# Autodesk Inventor assembly: Ribbon_Twitter
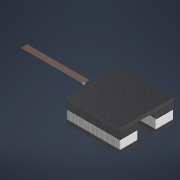
[picture p0: Inventor's stored thumbnail of the model, 180x180]
Saved by Autodesk Inventor 2022 (Build 260153070, 153G)
## iProperties
Created: 2022-02-01
Part Number: Ribbon_Twitter
Document SubType Name: Assembly
Designer: kalugin_a
Author: kalugin_a
## Documents named in this file (7)
- C:\Users\kalugin_a\Documents\Inventor\TUTO\MELAS\Workspace\Ribbon_Twitter.iam
- C:\Users\kalugin_a\Documents\Inventor\TUTO\MELAS\Workspace\NS.ipt
- C:\Users\kalugin_a\Documents\Inventor\TUTO\MELAS\Workspace\plate.ipt
- C:\Users\kalugin_a\Documents\Inventor\TUTO\MELAS\Workspace\Plate1.ipt
- C:\Users\kalugin_a\Documents\Inventor\TUTO\MELAS\Workspace\flange.ipt
- C:\Users\kalugin_a\Documents\Inventor\TUTO\MELAS\Workspace\Mwire.ipt
- C:\Users\kalugin_a\Documents\Inventor\TUTO\MELAS\Workspace\ribbon.ipt
## Components (11 placed, 6 different names)
1. NS:1 — Заподлицо:9, Заподлицо:10, Совмещение:5, Совмещение:7, Совмещение:8, Заподлицо:13, Заподлицо:14
2. NS:2 — Совмещение:6, Заподлицо:11, Заподлицо:12, Совмещение:9, Заподлицо:15, Заподлицо:16
3. plate:1 — Заподлицо:1, Заподлицо:2, Совмещение:1, Заподлицо:5, Заподлицо:6, Совмещение:3
4. Plate1:1 — Заподлицо:5, Заподлицо:6, Совмещение:3, Заподлицо:7, Совмещение:4, Заподлицо:8, Заподлицо:10
5. Plate1:2 — Заподлицо:1, Заподлицо:2, Совмещение:1, Заподлицо:3, Заподлицо:4, Совмещение:2, Заподлицо:12
6. Plate1:3 — Заподлицо:7, Совмещение:4, Заподлицо:8, Заподлицо:9, Совмещение:5
7. Plate1:4 — Заподлицо:3, Заподлицо:4, Совмещение:2, Совмещение:6, Заподлицо:11
8. flange:1 — Совмещение:7
9. Mwire:1 — Совмещение:8, Заподлицо:13, Заподлицо:14
10. Mwire:2 — Совмещение:9, Заподлицо:15, Заподлицо:16
11. ribbon:1
## Relationships (25: Flush 16, Mate 9)
- Заподлицо:1 [Flush]: plate:1 ↔ Plate1:2
- Заподлицо:2 [Flush]: plate:1 ↔ Plate1:2
- Совмещение:1 [Mate]: plate:1 ↔ Plate1:2
- Заподлицо:3 [Flush]: Plate1:2 ↔ Plate1:4
- Заподлицо:4 [Flush]: Plate1:2 ↔ Plate1:4
- Совмещение:2 [Mate]: Plate1:2 ↔ Plate1:4
- Заподлицо:5 [Flush]: plate:1 ↔ Plate1:1
- Заподлицо:6 [Flush]: plate:1 ↔ Plate1:1
- Совмещение:3 [Mate]: plate:1 ↔ Plate1:1
- Заподлицо:7 [Flush]: Plate1:1 ↔ Plate1:3
- Совмещение:4 [Mate]: Plate1:1 ↔ Plate1:3
- Заподлицо:8 [Flush]: Plate1:1 ↔ Plate1:3
- Заподлицо:9 [Flush]: NS:1 ↔ Plate1:3
- Заподлицо:10 [Flush]: NS:1 ↔ Plate1:1
- Совмещение:5 [Mate]: NS:1 ↔ Plate1:3
- Совмещение:6 [Mate]: NS:2 ↔ Plate1:4
- Заподлицо:11 [Flush]: NS:2 ↔ Plate1:4
- Заподлицо:12 [Flush]: NS:2 ↔ Plate1:2
- Совмещение:7 [Mate] (50 mm): NS:1 ↔ flange:1
- Совмещение:8 [Mate]: NS:1 ↔ Mwire:1
- Заподлицо:13 [Flush]: NS:1 ↔ Mwire:1
- Заподлицо:14 [Flush]: NS:1 ↔ Mwire:1
- Совмещение:9 [Mate]: NS:2 ↔ Mwire:2
- Заподлицо:15 [Flush]: NS:2 ↔ Mwire:2
- Заподлицо:16 [Flush]: NS:2 ↔ Mwire:2
